# Autodesk Inventor assembly: Assembly
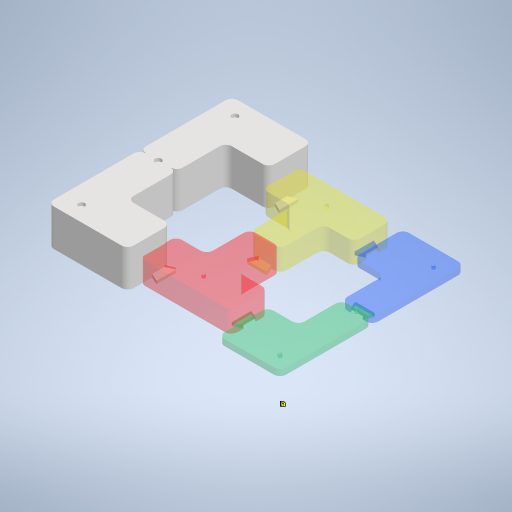
[picture p0: Inventor's stored thumbnail of the model, 512x512]
Saved by Autodesk Inventor 2024 (Build 280153000, 153)
## iProperties
Created: 2024-03-01
Part Number: Assembly
Document SubType Name: Assembly
Designer: laura
Author: laura
## Documents named in this file (7)
- C:\Users\laura\OneDrive\Dokumenter\GitHub\2_Semesterprojekt\inventor\Build filer plade\Assembly.iam
- C:\Users\laura\OneDrive\Dokumenter\GitHub\2_Semesterprojekt\inventor\Build filer plade\Area nh.ipt
- C:\Users\laura\OneDrive\Dokumenter\GitHub\2_Semesterprojekt\inventor\Build filer plade\Area nv.ipt
- C:\Users\laura\OneDrive\Dokumenter\GitHub\2_Semesterprojekt\inventor\Build filer plade\Area mh.ipt
- C:\Users\laura\OneDrive\Dokumenter\GitHub\2_Semesterprojekt\inventor\Build filer plade\Area mv.ipt
- C:\Users\laura\OneDrive\Dokumenter\GitHub\2_Semesterprojekt\inventor\Build filer plade\Area øh.ipt
- C:\Users\laura\OneDrive\Dokumenter\GitHub\2_Semesterprojekt\inventor\Build filer plade\Area øv.ipt
## Components (6 placed, 6 different names)
1. Area nh:1 — Slider:2, Rigid:2
2. Area nv:1 — Rigid:2
3. Area mh:1 — Slider:2, Slider:3
4. Area mv:1
5. Area øh:1 — Slider:3, Slider:4
6. Area øv:1 — Slider:4
## Relationships (4: TranslationJoint 3, WeldJoint 1)
- Slider:2 [TranslationJoint]: Area nh:1 ↔ Area mh:1
- Slider:3 [TranslationJoint]: Area mh:1 ↔ Area øh:1
- Rigid:2 [WeldJoint]: Area nh:1 ↔ Area nv:1
- Slider:4 [TranslationJoint]: Area øh:1 ↔ Area øv:1
